# Autodesk Inventor assembly: 76. Крышка верхняя в сборе
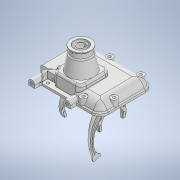
[picture p0: Inventor's stored thumbnail of the model, 180x180]
Saved by Autodesk Inventor 2021 (Build 250183000, 183)
## iProperties
Created: 2021-04-09
Part Number: 76. Крышка верхняя в сборе
Document SubType Name: Assembly
Designer: Данил
Author: Данил
## Documents named in this file (23)
- C:\Users\Данил\Desktop\Коробка передач\Детали\76. Крышка верхняя в сборе.iam
- C:\Users\Данил\Desktop\Коробка передач\Детали\77. Крышка верхняя.ipt
- C:\Users\Данил\Desktop\Коробка передач\Детали\76. Шарик фиксатора.ipt
- C:\Users\Данил\Desktop\Коробка передач\Детали\405. Пружина стопорного шарика (нагрузка).ipt
- C:\Users\Данил\Desktop\Коробка передач\Детали\79. Вилка первой и второй передач.ipt
- C:\Users\Данил\Desktop\Коробка передач\Детали\76. Стопор.ipt
- C:\Users\Данил\Desktop\Коробка передач\Детали\76. Штифт.ipt
- C:\Users\Данил\Desktop\Коробка передач\Детали\80. Пружина рычага (свободна).ipt
- C:\Users\Данил\Desktop\Коробка передач\Детали\78. Головка штока первой и второй передач.ipt
- C:\Users\Данил\Desktop\Коробка передач\Детали\79. Головка заднего хода в сборе.iam
- C:\Users\Данил\Desktop\Коробка передач\Детали\78. Вилка третьей и четвертой передачи.ipt
- C:\Users\Данил\Desktop\Коробка передач\Детали\79. Вилка заднего хода.ipt
- C:\Users\Данил\Desktop\Коробка передач\Детали\80. Шток заднего хода.ipt
- C:\Users\Данил\Desktop\Коробка передач\Детали\79. Шток третьей и четвертой передач.ipt
- C:\Users\Данил\Desktop\Коробка передач\Детали\80. Шток первой и второй передач.ipt
- C:\Users\Данил\Desktop\Коробка передач\Детали\68. Заглушка.ipt
- C:\Users\Данил\Desktop\Коробка передач\Детали\80. Плунжер стопорный штоков.ipt
- C:\Users\Данил\Desktop\Коробка передач\Детали\78. Стопорный палец.ipt
- C:\Users\Данил\Desktop\Коробка передач\Детали\76. Заглушка.ipt
- C:\Users\Данил\Desktop\Коробка передач\Детали\76. Стопор первой и второй передач.ipt
- C:\Users\Данил\Desktop\Коробка передач\Детали\76. Стопор заднего хода.ipt
- C:\Users\Данил\Documents\Inventor\Content Center Files\R2021\ru-RU\Bolt 4A GOST 15591-70\Болт 4A M10×16 ГОСТ 15591-70.ipt
- C:\Users\Данил\Documents\Inventor\Content Center Files\R2021\ru-RU\GOST 397-79\Шплинт 1,2x20 ГОСТ 397-79.ipt
## Components (32 placed, 22 different names)
1. 77. Крышка верхняя:1 — Совмещение:1, Совмещение:2, Заподлицо:1, Совмещение:3, Совмещение:4, Совмещение:6, Совмещение:10, Совмещение:11, Совмещение:12, Совмещение:13, Совмещение:14, Совмещение:15, Совмещение:16, Совмещение:17, Угол:1, Угол:2, Угол:3, Совмещение:20, Совмещение:21, Заподлицо:2, Совмещение:22, Заподлицо:3, Заподлицо:4, Заподлицо:5, Совмещение:23, Заподлицо:6, Совмещение:24, Совмещение:25, Совмещение:26, Заподлицо:7, Заподлицо:8, Заподлицо:9, Совмещение:28, Угол:4, Угол:5
2. 79. Вилка первой и второй передач:1 — Совмещение:42, Угол:5, Совмещение:43, Совмещение:44, Совмещение:49
3. 76. Стопор:1 — Совмещение:35, Заподлицо:13
4. 76. Штифт:1 — Совмещение:3, Совмещение:5
5. 76. Штифт:2 — Совмещение:4, Совмещение:5, Совмещение:6
6. 80. Пружина рычага (свободна):1 — Совмещение:1, Совмещение:2, Заподлицо:1
7. 78. Головка штока первой и второй передач:1 — Совмещение:33, Совмещение:37, Совмещение:38
8. 79. Головка заднего хода в сборе:1 [sub-assembly] — Совмещение:32, Заподлицо:11, Совмещение:40, Совмещение:41
9. 78. Вилка третьей и четвертой передачи:1 — Совмещение:30, Угол:4, Заподлицо:11, Совмещение:45, Касательность:2
10. 79. Вилка заднего хода:1 — Совмещение:29, Совмещение:34, Заподлицо:13
11. 80. Шток заднего хода:1 — Совмещение:17, Угол:3, Заподлицо:5, Совмещение:29, Совмещение:32, Совмещение:34, Совмещение:35, Совмещение:39, Совмещение:40
12. 79. Шток третьей и четвертой передач:1 — Совмещение:16, Угол:2, Заподлицо:4, Совмещение:27, Совмещение:30
13. 80. Шток первой и второй передач:1 — Совмещение:15, Угол:1, Совмещение:18, Заподлицо:3, Совмещение:33, Совмещение:36, Совмещение:42, Совмещение:43
14. 68. Заглушка:1 — Совмещение:23, Заподлицо:6
15. 80. Плунжер стопорный штоков:1 — Совмещение:18, Совмещение:19, Совмещение:20, Заподлицо:2
16. 80. Плунжер стопорный штоков:2 — Совмещение:19, Совмещение:21, Совмещение:22
17. 78. Стопорный палец:1 — Совмещение:27, Совмещение:28
18. 76. Заглушка:1 — Совмещение:25, Заподлицо:8
19. 76. Заглушка:2 — Совмещение:24, Заподлицо:9
20. 76. Заглушка:3 — Совмещение:26, Заподлицо:7
21. 76. Стопор первой и второй передач:1 — Совмещение:36, Совмещение:37, Совмещение:38
22. 76. Стопор заднего хода:1 — Совмещение:39, Совмещение:41
23. Болт 4A ГОСТ 15591-70 M10×16:1 — Совмещение:44, Совмещение:46, Совмещение:48, Совмещение:49
24. Болт 4A ГОСТ 15591-70 M10×16:2 — Совмещение:45, Совмещение:50, Совмещение:51, Касательность:2
25. Шплинт ГОСТ 397-79 1,2 x  20:1 — Совмещение:46, Совмещение:48
26. Шплинт ГОСТ 397-79 1,2 x  20:2 — Совмещение:50, Совмещение:51
27. 405. Пружина стопорного шарика (нагрузка):3 — Совмещение:11, Совмещение:12, Совмещение:14, Касательность:1
28. 76. Шарик фиксатора:1 — Совмещение:10, Совмещение:13, Касательность:1
29. 405. Пружина стопорного шарика (нагрузка):4
30. 76. Шарик фиксатора:2
31. 405. Пружина стопорного шарика (нагрузка):5
32. 76. Шарик фиксатора:3
## Component patterns: (3 elements, first: 405. Пружина стопорного шарика (нагрузка):3 + 76. Шарик фиксатора:1)
## Relationships (64: Mate 46, Flush 11, Angle 5, Tangent 2)
- Совмещение:1 [Mate]: 77. Крышка верхняя:1 ↔ 80. Пружина рычага (свободна):1
- Совмещение:2 [Mate]: 77. Крышка верхняя:1 ↔ 80. Пружина рычага (свободна):1
- Заподлицо:1 [Flush]: 77. Крышка верхняя:1 ↔ 80. Пружина рычага (свободна):1
- Совмещение:3 [Mate]: 77. Крышка верхняя:1 ↔ 76. Штифт:1
- Совмещение:4 [Mate]: 77. Крышка верхняя:1 ↔ 76. Штифт:2
- Совмещение:5 [Mate] (33 mm): 76. Штифт:1 ↔ 76. Штифт:2
- Совмещение:6 [Mate] (-16.5 mm): 77. Крышка верхняя:1 ↔ 76. Штифт:2
- Совмещение:10 [Mate] (28 mm): 77. Крышка верхняя:1 ↔ 76. Шарик фиксатора:1
- Совмещение:11 [Mate] (28 mm): 77. Крышка верхняя:1 ↔ 405. Пружина стопорного шарика (нагрузка):3
- Совмещение:12 [Mate] (-52 mm): 77. Крышка верхняя:1 ↔ 405. Пружина стопорного шарика (нагрузка):3
- Совмещение:13 [Mate] (-52 mm): 77. Крышка верхняя:1 ↔ 76. Шарик фиксатора:1
- Совмещение:14 [Mate]: 77. Крышка верхняя:1 ↔ 405. Пружина стопорного шарика (нагрузка):3
- Касательность:1 [Tangent]: 405. Пружина стопорного шарика (нагрузка):3 ↔ 76. Шарик фиксатора:1
- Совмещение:15 [Mate]: 77. Крышка верхняя:1 ↔ 80. Шток первой и второй передач:1
- Совмещение:16 [Mate]: 77. Крышка верхняя:1 ↔ 79. Шток третьей и четвертой передач:1
- Совмещение:17 [Mate]: 77. Крышка верхняя:1 ↔ 80. Шток заднего хода:1
- Угол:1 [Angle] (0 deg): 77. Крышка верхняя:1 ↔ 80. Шток первой и второй передач:1
- Угол:2 [Angle] (0 deg): 77. Крышка верхняя:1 ↔ 79. Шток третьей и четвертой передач:1
- Угол:3 [Angle] (0 deg): 77. Крышка верхняя:1 ↔ 80. Шток заднего хода:1
- Совмещение:18 [Mate]: 80. Шток первой и второй передач:1 ↔ 80. Плунжер стопорный штоков:1
- Совмещение:19 [Mate]: 80. Плунжер стопорный штоков:1 ↔ 80. Плунжер стопорный штоков:2
- Совмещение:20 [Mate]: 77. Крышка верхняя:1 ↔ 80. Плунжер стопорный штоков:1
- Совмещение:21 [Mate]: 77. Крышка верхняя:1 ↔ 80. Плунжер стопорный штоков:2
- Заподлицо:2 [Flush] (-14 mm): 77. Крышка верхняя:1 ↔ 80. Плунжер стопорный штоков:1
- Совмещение:22 [Mate] (14 mm): 77. Крышка верхняя:1 ↔ 80. Плунжер стопорный штоков:2
- Заподлицо:3 [Flush] (-10 mm): 77. Крышка верхняя:1 ↔ 80. Шток первой и второй передач:1
- Заподлицо:4 [Flush] (-3.7 mm): 77. Крышка верхняя:1 ↔ 79. Шток третьей и четвертой передач:1
- Заподлицо:5 [Flush] (11.5 mm): 77. Крышка верхняя:1 ↔ 80. Шток заднего хода:1
- Совмещение:23 [Mate]: 77. Крышка верхняя:1 ↔ 68. Заглушка:1
- Заподлицо:6 [Flush]: 77. Крышка верхняя:1 ↔ 68. Заглушка:1
- Совмещение:24 [Mate]: 77. Крышка верхняя:1 ↔ 76. Заглушка:2
- Совмещение:25 [Mate]: 77. Крышка верхняя:1 ↔ 76. Заглушка:1
- Совмещение:26 [Mate]: 77. Крышка верхняя:1 ↔ 76. Заглушка:3
- Заподлицо:7 [Flush]: 77. Крышка верхняя:1 ↔ 76. Заглушка:3
- Заподлицо:8 [Flush]: 77. Крышка верхняя:1 ↔ 76. Заглушка:1
- Заподлицо:9 [Flush]: 77. Крышка верхняя:1 ↔ 76. Заглушка:2
- Совмещение:27 [Mate]: 79. Шток третьей и четвертой передач:1 ↔ 78. Стопорный палец:1
- Совмещение:28 [Mate]: 77. Крышка верхняя:1 ↔ 78. Стопорный палец:1
- Совмещение:29 [Mate]: 79. Вилка заднего хода:1 ↔ 80. Шток заднего хода:1
- Совмещение:30 [Mate]: 78. Вилка третьей и четвертой передачи:1 ↔ 79. Шток третьей и четвертой передач:1
- Совмещение:32 [Mate]: 79. Головка заднего хода в сборе:1 ↔ 80. Шток заднего хода:1
- Совмещение:33 [Mate]: 78. Головка штока первой и второй передач:1 ↔ 80. Шток первой и второй передач:1
- Угол:4 [Angle] (0 deg): 77. Крышка верхняя:1 ↔ 78. Вилка третьей и четвертой передачи:1
- Заподлицо:11 [Flush]: 79. Головка заднего хода в сборе:1 ↔ 78. Вилка третьей и четвертой передачи:1
- Совмещение:34 [Mate]: 79. Вилка заднего хода:1 ↔ 80. Шток заднего хода:1
- Совмещение:35 [Mate]: 76. Стопор:1 ↔ 80. Шток заднего хода:1
- Заподлицо:13 [Flush]: 76. Стопор:1 ↔ 79. Вилка заднего хода:1
- Совмещение:36 [Mate]: 80. Шток первой и второй передач:1 ↔ 76. Стопор первой и второй передач:1
- Совмещение:37 [Mate]: 78. Головка штока первой и второй передач:1 ↔ 76. Стопор первой и второй передач:1
- Совмещение:38 [Mate]: 78. Головка штока первой и второй передач:1 ↔ 76. Стопор первой и второй передач:1
- Совмещение:39 [Mate]: 80. Шток заднего хода:1 ↔ 76. Стопор заднего хода:1
- Совмещение:40 [Mate]: 79. Головка заднего хода в сборе:1 ↔ 80. Шток заднего хода:1
- Совмещение:41 [Mate] (-12 mm): 79. Головка заднего хода в сборе:1 ↔ 76. Стопор заднего хода:1
- Совмещение:42 [Mate]: 79. Вилка первой и второй передач:1 ↔ 80. Шток первой и второй передач:1
- Угол:5 [Angle] (0 deg): 77. Крышка верхняя:1 ↔ 79. Вилка первой и второй передач:1
- Совмещение:43 [Mate]: 79. Вилка первой и второй передач:1 ↔ 80. Шток первой и второй передач:1
- Совмещение:44 [Mate]: 79. Вилка первой и второй передач:1 ↔ Болт 4A ГОСТ 15591-70 M10×16:1
- Совмещение:45 [Mate]: 78. Вилка третьей и четвертой передачи:1 ↔ Болт 4A ГОСТ 15591-70 M10×16:2
- Совмещение:46 [Mate]: Болт 4A ГОСТ 15591-70 M10×16:1 ↔ Шплинт ГОСТ 397-79 1,2 x  20:1
- Совмещение:48 [Mate] (-8 mm): Болт 4A ГОСТ 15591-70 M10×16:1 ↔ Шплинт ГОСТ 397-79 1,2 x  20:1
- Совмещение:49 [Mate]: 79. Вилка первой и второй передач:1 ↔ Болт 4A ГОСТ 15591-70 M10×16:1
- Совмещение:50 [Mate]: Болт 4A ГОСТ 15591-70 M10×16:2 ↔ Шплинт ГОСТ 397-79 1,2 x  20:2
- Совмещение:51 [Mate] (-8 mm): Болт 4A ГОСТ 15591-70 M10×16:2 ↔ Шплинт ГОСТ 397-79 1,2 x  20:2
- Касательность:2 [Tangent]: 78. Вилка третьей и четвертой передачи:1 ↔ Болт 4A ГОСТ 15591-70 M10×16:2
